# Autodesk Inventor assembly: XY Drive Subassy
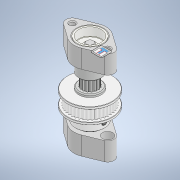
[picture p0: Inventor's stored thumbnail of the model, 180x180]
Saved by Autodesk Inventor 2022 (Build 260153000, 153)
## iProperties
Created: 2021-10-06
Part Number: XY Drive Subassy
Document SubType Name: Assembly
Designer: nicol
Author: nicol
## Documents named in this file (8)
- Y:\Projects\Bibble0\XY Drive Subassy.iam
- Y:\Projects\Bibble0\Bearings\625 Bearing.ipt
- Y:\Projects\Bibble0\3D printed\XY Drive Bearing Holder.ipt
- Y:\Projects\Bibble0\Hardware\GT2 Pulley 16T.ipt
- Y:\Projects\Bibble0\Hardware\5 x 50mm Shaft.ipt
- Y:\Projects\Bibble0\3D printed\Bearing Retaining Ring.ipt
- Y:\Projects\Bibble0\Hardware\GT2 40T 5mm Bore.ipt
- Y:\Projects\Bibble0\5mmx3mm spacer.ipt
## Components (12 placed, 7 different names)
1. 625 Bearing:1 — Insert:7, Insert:13, Insert:15, Insert:16
2. 625 Bearing:2 — Insert:8, Insert:11, Insert:14
3. XY Drive Bearing Holder:1 — Mate:1, Insert:14
4. XY Drive Bearing Holder:2 — Mate:1, Insert:15
5. GT2 Pulley 16T:1 — Insert:4
6. GT2 Pulley 16T:2 — Insert:4, Insert:9, Insert:10
7. 5 x 50mm Shaft:1 — Insert:16
8. Bearing Retaining Ring:1 — Insert:7
9. Bearing Retaining Ring:2 — Insert:8
10. GT2 40T 5mm Bore:1 — Insert:9, Insert:12
11. 5mmx3mm spacer:1 — Insert:10, Insert:11
12. 5mmx3mm spacer:2 — Insert:12, Insert:13
## Relationships (12: Insert 11, Mate 1)
- Insert:4: GT2 Pulley 16T:1 ↔ GT2 Pulley 16T:2
- Insert:7: 625 Bearing:1 ↔ Bearing Retaining Ring:1
- Insert:8: 625 Bearing:2 ↔ Bearing Retaining Ring:2
- Mate:1: XY Drive Bearing Holder:1 ↔ XY Drive Bearing Holder:2
- Insert:9: GT2 Pulley 16T:2 ↔ GT2 40T 5mm Bore:1
- Insert:10: GT2 Pulley 16T:2 ↔ 5mmx3mm spacer:1
- Insert:11: 625 Bearing:2 ↔ 5mmx3mm spacer:1
- Insert:12: GT2 40T 5mm Bore:1 ↔ 5mmx3mm spacer:2
- Insert:13: 625 Bearing:1 ↔ 5mmx3mm spacer:2
- Insert:14: 625 Bearing:2 ↔ XY Drive Bearing Holder:1
- Insert:15: 625 Bearing:1 ↔ XY Drive Bearing Holder:2
- Insert:16: 625 Bearing:1 ↔ 5 x 50mm Shaft:1
